# Autodesk Inventor assembly: DB_DriveBaseSquare_AM14U2
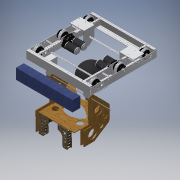
[picture p0: Inventor's stored thumbnail of the model, 180x180]
Saved by Autodesk Inventor 2016 (Build 200138000, 138)
## iProperties
Category: Drive Base
Company: Autodesk Inc.
Created: 2014-12-16
Part Number: DB_DriveBaseSquare_AM14U2
Document SubType Name: Assembly
Designer: Autodesk Inc.
Catalog Web Link: andymark.com
Vendor: Andy Mark Inc.
Author: Autodesk Inc.
## Documents named in this file (14)
- C:\Users\ares-b02\Documents\FRC 2016 Robot\DB_DriveBaseSquare_AM14U2.iam
- C:\Users\ares-b02\Documents\FRC 2015 Parts\Drive Base\Drive Base\Parts\AM14U2 Half Square.iam
- C:\Users\ares-b02\Documents\FRC 2016 Robot\Cote droit Rammasse-Balle.ipt
- C:\Users\ares-b02\Documents\FRC 2016 Robot\Cote gauche Rammasse-Balle.ipt
- C:\Users\ares-b02\Documents\FRC 2016 Robot\Devant - Bas Rammasse-Balle.ipt
- C:\Users\ares-b02\Documents\FRC 2016 Robot\Part9.ipt
- C:\Users\ares-b02\Documents\FRC 2016 Robot\Braquet Rammasse-Balle.ipt
- C:\Users\ares-b02\Documents\Inventor\Content Center Files\R2016\en-US\ISO 7092\ISO 7092 - ST 8 - 140 HV.ipt
- C:\Users\ares-b02\Documents\FRC 2016 Robot\Devant - Haut Rammasse-Balle.ipt
- C:\Users\ares-b02\Documents\FRC 2016 Robot\balle.ipt
- C:\Users\ares-b02\Documents\FRC 2016 Robot\Bumper.ipt
- C:\Users\ares-b02\Documents\FRC 2016 Robot\arm droit.ipt
- C:\Users\ares-b02\Documents\FRC 2016 Robot\spacer.ipt
- C:\Users\ares-b02\Documents\FRC 2016 Robot\arm gauche.ipt
## Components (52 placed, 14 different names)
1. AM14U2 Half Square_1 [sub-assembly] — Insert:1, Mate:1, Mate:4, Mate:6, Mate:18, Mate:19
2. AM14U2 Half Square_2 [sub-assembly] — Insert:1, Mate:2, Mate:3, Mate:5
3. Cote droit Rammasse-Balle:1 — Mate:8, Mate:13, Flush:1, Flush:4, Flush:5, Mate:20, Flush:7, Mate:68, Flush:9
4. Cote gauche Rammasse-Balle:1 — Mate:14, Mate:15, Flush:1, Flush:2, Mate:61, Mate:63, Mate:67, Flush:8
5. Devant - Bas Rammasse-Balle:1 — Flush:2, Flush:4, Flush:5, Mate:21, Mate:64, Mate:103, Mate:104
6. Part9:1 — Mate:7, Mate:8, Mate:9, Mate:11, Mate:14, Mate:65, Mate:66
7. Braquet Rammasse-Balle:1 — Mate:2, Mate:3, Mate:5, Mate:10
8. Braquet Rammasse-Balle:2 — Mate:1, Mate:4, Mate:6, Mate:7, Mate:12
9. ISO 7092 ST 8 - 140 HV:1 — Mate:9, Mate:10, Mate:13
10. ISO 7092 ST 8 - 140 HV:2 — Mate:11, Mate:12, Mate:15
11. Devant - Haut Rammasse-Balle:1 — Mate:61, Mate:63, Mate:64
12. balle:1
13. Bumper:1 — Mate:18, Mate:19
14. arm droit:1 — Mate:40, Mate:59
15. arm droit:2 — Mate:20, Mate:21, Flush:7, Mate:22, Mate:24, Mate:25, Mate:26, Mate:27, Mate:28, Mate:29, Mate:30, Mate:32, Mate:33, Mate:34, Mate:35, Mate:36, Mate:37, Mate:38, Mate:39, Mate:40, Mate:42, Mate:43, Mate:44, Mate:45, Mate:46, Mate:47, Mate:49, Mate:50, Mate:51, Mate:52, Mate:53, Mate:54, Mate:55, Mate:56, Mate:57, Mate:58, Flush:105, Mate:104
16. spacer:1 — Mate:38, Mate:52
17. spacer:2 — Mate:34, Mate:44
18. spacer:3 — Mate:35, Mate:45
19. spacer:4 — Mate:37, Mate:47
20. spacer:5 — Mate:36, Mate:46
21. spacer:6 — Mate:39, Mate:55
22. spacer:7 — Mate:33, Mate:43
23. spacer:8 — Mate:32, Mate:42
24. spacer:10 — Mate:30, Mate:57, Mate:59
25. spacer:11 — Mate:29, Mate:58
26. spacer:12 — Mate:28, Mate:54
27. spacer:13 — Mate:27, Mate:53
28. spacer:14 — Mate:26, Mate:51
29. spacer:15 — Mate:25, Mate:50
30. spacer:16 — Mate:24, Mate:49
31. spacer:18 — Mate:22, Mate:56
32. spacer:22 — Mate:83, Mate:92, Mate:100
33. spacer:23 — Mate:82, Mate:93
34. spacer:24 — Mate:84, Mate:98
35. spacer:25 — Mate:81, Mate:94
36. spacer:26 — Mate:80, Mate:95, Mate:102
37. spacer:27 — Mate:76, Mate:96, Mate:101
38. spacer:28 — Mate:79, Mate:99
39. spacer:29 — Mate:77, Mate:97
40. spacer:30 — Mate:75, Mate:91
41. spacer:31 — Mate:74, Mate:90
42. spacer:32 — Mate:73, Mate:89
43. spacer:33 — Mate:72, Mate:88
44. spacer:34 — Mate:71, Mate:87
45. spacer:35 — Mate:70, Mate:86
46. spacer:36 — Mate:69, Mate:85
47. arm gauche:1 — Mate:100, Mate:101, Mate:102, Flush:105
48. arm gauche:2 — Mate:69, Mate:70, Mate:71, Mate:72, Mate:73, Mate:74, Mate:75, Mate:76, Mate:77, Mate:79, Mate:80, Mate:81, Mate:82, Mate:83, Mate:84, Mate:85, Mate:86, Mate:87, Mate:88, Mate:89, Mate:90, Mate:91, Mate:92, Mate:93, Mate:94, Mate:95, Mate:96, Mate:97, Mate:98, Mate:99, Mate:103
49. Cote droit Rammasse-Balle:2 — Mate:66, Mate:68, Flush:9
50. Cote gauche Rammasse-Balle:2 — Mate:65, Mate:67, Flush:8
51. Braquet Rammasse-Balle:3
52. Braquet Rammasse-Balle:4
## Relationships (104: Mate 95, Flush 8, Insert 1)
- Insert:1: AM14U2 Half Square_1 ↔ AM14U2 Half Square_2
- Mate:1: AM14U2 Half Square_1 ↔ Braquet Rammasse-Balle:2
- Mate:2: AM14U2 Half Square_2 ↔ Braquet Rammasse-Balle:1
- Mate:3: AM14U2 Half Square_2 ↔ Braquet Rammasse-Balle:1
- Mate:4: AM14U2 Half Square_1 ↔ Braquet Rammasse-Balle:2
- Mate:5: AM14U2 Half Square_2 ↔ Braquet Rammasse-Balle:1
- Mate:6: AM14U2 Half Square_1 ↔ Braquet Rammasse-Balle:2
- Mate:7: Part9:1 ↔ Braquet Rammasse-Balle:2
- Mate:8: Cote droit Rammasse-Balle:1 ↔ Part9:1
- Mate:9: Part9:1 ↔ ISO 7092 ST 8 - 140 HV:1
- Mate:10: Braquet Rammasse-Balle:1 ↔ ISO 7092 ST 8 - 140 HV:1
- Mate:11: Part9:1 ↔ ISO 7092 ST 8 - 140 HV:2
- Mate:12: Braquet Rammasse-Balle:2 ↔ ISO 7092 ST 8 - 140 HV:2
- Mate:13: Cote droit Rammasse-Balle:1 ↔ ISO 7092 ST 8 - 140 HV:1
- Mate:14: Cote gauche Rammasse-Balle:1 ↔ Part9:1
- Mate:15: Cote gauche Rammasse-Balle:1 ↔ ISO 7092 ST 8 - 140 HV:2
- Flush:1: Cote droit Rammasse-Balle:1 ↔ Cote gauche Rammasse-Balle:1
- Flush:2 (6.35 mm): Cote gauche Rammasse-Balle:1 ↔ Devant - Bas Rammasse-Balle:1
- Flush:4: Cote droit Rammasse-Balle:1 ↔ Devant - Bas Rammasse-Balle:1
- Flush:5: Cote droit Rammasse-Balle:1 ↔ Devant - Bas Rammasse-Balle:1
- Mate:18 (31.75 mm): AM14U2 Half Square_1 ↔ Bumper:1
- Mate:19 (20 mm): AM14U2 Half Square_1 ↔ Bumper:1
- Mate:20: Cote droit Rammasse-Balle:1 ↔ arm droit:2
- Mate:21: Devant - Bas Rammasse-Balle:1 ↔ arm droit:2
- Flush:7: Cote droit Rammasse-Balle:1 ↔ arm droit:2
- Mate:22: arm droit:2 ↔ spacer:18
- Mate:24: arm droit:2 ↔ spacer:16
- Mate:25: arm droit:2 ↔ spacer:15
- Mate:26: arm droit:2 ↔ spacer:14
- Mate:27: arm droit:2 ↔ spacer:13
- Mate:28: arm droit:2 ↔ spacer:12
- Mate:29: arm droit:2 ↔ spacer:11
- Mate:30: arm droit:2 ↔ spacer:10
- Mate:32: arm droit:2 ↔ spacer:8
- Mate:33: arm droit:2 ↔ spacer:7
- Mate:34: arm droit:2 ↔ spacer:2
- Mate:35: arm droit:2 ↔ spacer:3
- Mate:36: arm droit:2 ↔ spacer:5
- Mate:37: arm droit:2 ↔ spacer:4
- Mate:38: arm droit:2 ↔ spacer:1
- Mate:39: arm droit:2 ↔ spacer:6
- Mate:40 (38.1 mm): arm droit:1 ↔ arm droit:2
- Mate:42: arm droit:2 ↔ spacer:8
- Mate:43: arm droit:2 ↔ spacer:7
- Mate:44: arm droit:2 ↔ spacer:2
- Mate:45: arm droit:2 ↔ spacer:3
- Mate:46: arm droit:2 ↔ spacer:5
- Mate:47: arm droit:2 ↔ spacer:4
- Mate:49: arm droit:2 ↔ spacer:16
- Mate:50: arm droit:2 ↔ spacer:15
- Mate:51: arm droit:2 ↔ spacer:14
- Mate:52: arm droit:2 ↔ spacer:1
- Mate:53: arm droit:2 ↔ spacer:13
- Mate:54: arm droit:2 ↔ spacer:12
- Mate:55: arm droit:2 ↔ spacer:6
- Mate:56: arm droit:2 ↔ spacer:18
- Mate:57: arm droit:2 ↔ spacer:10
- Mate:58: arm droit:2 ↔ spacer:11
- Mate:59: arm droit:1 ↔ spacer:10
- Mate:61: Cote gauche Rammasse-Balle:1 ↔ Devant - Haut Rammasse-Balle:1
- Mate:63: Cote gauche Rammasse-Balle:1 ↔ Devant - Haut Rammasse-Balle:1
- Mate:64: Devant - Bas Rammasse-Balle:1 ↔ Devant - Haut Rammasse-Balle:1
- Mate:65: Part9:1 ↔ Cote gauche Rammasse-Balle:2
- Mate:66: Part9:1 ↔ Cote droit Rammasse-Balle:2
- Mate:67 (25.4 mm): Cote gauche Rammasse-Balle:1 ↔ Cote gauche Rammasse-Balle:2
- Flush:8: Cote gauche Rammasse-Balle:1 ↔ Cote gauche Rammasse-Balle:2
- Mate:68 (25.4 mm): Cote droit Rammasse-Balle:1 ↔ Cote droit Rammasse-Balle:2
- Flush:9: Cote droit Rammasse-Balle:1 ↔ Cote droit Rammasse-Balle:2
- Mate:69: spacer:36 ↔ arm gauche:2
- Mate:70: spacer:35 ↔ arm gauche:2
- Mate:71: spacer:34 ↔ arm gauche:2
- Mate:72: spacer:33 ↔ arm gauche:2
- Mate:73: spacer:32 ↔ arm gauche:2
- Mate:74: spacer:31 ↔ arm gauche:2
- Mate:75: spacer:30 ↔ arm gauche:2
- Mate:76: spacer:27 ↔ arm gauche:2
- Mate:77: spacer:29 ↔ arm gauche:2
- Mate:79: spacer:28 ↔ arm gauche:2
- Mate:80: spacer:26 ↔ arm gauche:2
- Mate:81: spacer:25 ↔ arm gauche:2
- Mate:82: spacer:23 ↔ arm gauche:2
- Mate:83: spacer:22 ↔ arm gauche:2
- Mate:84: spacer:24 ↔ arm gauche:2
- Mate:85: spacer:36 ↔ arm gauche:2
- Mate:86: spacer:35 ↔ arm gauche:2
- Mate:87: spacer:34 ↔ arm gauche:2
- Mate:88: spacer:33 ↔ arm gauche:2
- Mate:89: spacer:32 ↔ arm gauche:2
- Mate:90: spacer:31 ↔ arm gauche:2
- Mate:91: spacer:30 ↔ arm gauche:2
- Mate:92: spacer:22 ↔ arm gauche:2
- Mate:93: spacer:23 ↔ arm gauche:2
- Mate:94: spacer:25 ↔ arm gauche:2
- Mate:95: spacer:26 ↔ arm gauche:2
- Mate:96: spacer:27 ↔ arm gauche:2
- Mate:97: spacer:29 ↔ arm gauche:2
- Mate:98: spacer:24 ↔ arm gauche:2
- Mate:99: spacer:28 ↔ arm gauche:2
- Mate:100: spacer:22 ↔ arm gauche:1
- Mate:101: spacer:27 ↔ arm gauche:1
- Mate:102: spacer:26 ↔ arm gauche:1
- Mate:103 (6.35 mm): Devant - Bas Rammasse-Balle:1 ↔ arm gauche:2
- Flush:105: arm droit:2 ↔ arm gauche:1
- Mate:104: Devant - Bas Rammasse-Balle:1 ↔ arm droit:2
